# Autodesk Inventor assembly: s-assy-unit-planet_gear
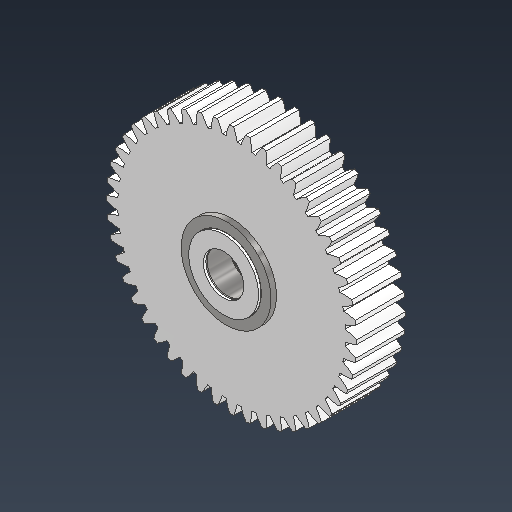
[picture p0: Inventor's stored thumbnail of the model, 512x512]
Saved by Autodesk Inventor 2021 (Build 250183000, 183)
## iProperties
Created: 2021-07-12
Part Number: s-assy-unit-planet_gear
Document SubType Name: Assembly
Designer: yuta0
Author: yuta0
## Documents named in this file (4)
- C:\Users\yuta0\Desktop\catchrobo_robot\s-assy-unit-planet_gear.iam
- C:\Users\yuta0\Desktop\catchrobo_robot\base32.ipt
- C:\Users\yuta0\Desktop\catchrobo_robot\FL688ZZ.ipt
- C:\Users\yuta0\Desktop\catchrobo_robot\base34.ipt
## Components (5 placed, 3 different names)
1. base32:1 — メイト:1, メイト:2, メイト:3, メイト:4
2. FL688ZZ:1 — メイト:1, メイト:2, メイト:7, メイト:8
3. FL688ZZ:2 — メイト:3, メイト:4, メイト:5, メイト:6
4. base34:1 — メイト:5, メイト:6
5. base34:2 — メイト:7, メイト:8
## Relationships (8: Mate 8)
- メイト:1 [Mate]: base32:1 ↔ FL688ZZ:1
- メイト:2 [Mate]: base32:1 ↔ FL688ZZ:1
- メイト:3 [Mate]: base32:1 ↔ FL688ZZ:2
- メイト:4 [Mate]: base32:1 ↔ FL688ZZ:2
- メイト:5 [Mate]: FL688ZZ:2 ↔ base34:1
- メイト:6 [Mate]: FL688ZZ:2 ↔ base34:1
- メイト:7 [Mate]: FL688ZZ:1 ↔ base34:2
- メイト:8 [Mate]: FL688ZZ:1 ↔ base34:2
